# Autodesk Inventor assembly: Assembly
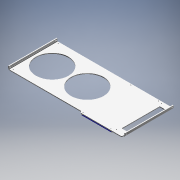
[picture p0: Inventor's stored thumbnail of the model, 180x180]
Saved by Autodesk Inventor 2018 (Build 220112000, 112)
## iProperties
Created: 2020-03-12
Part Number: Assembly
Document SubType Name: Assembly
Designer: tomah
Author: tomah
## Documents named in this file (3)
- E:\github projects\RSV-L4500 Console Hardware\Hardware\Assembly.iam
- E:\github projects\RSV-L4500 Console Hardware\Hardware\Plate.ipt
- E:\github projects\RSV-L4500 Console Hardware\Hardware\libraries\nextion-7\nextion_7inch.ipt
## Components (2 placed, 2 different names)
1. Plate:1 — Insert:1, Angle:1
2. nextion_7inch:1 — Insert:1, Angle:1
## Relationships (2: Insert 1, Angle 1)
- Insert:1 (3.175 mm): Plate:1 ↔ nextion_7inch:1
- Angle:1 (0 deg): Plate:1 ↔ nextion_7inch:1
